# Autodesk Inventor assembly: Ensamble Herramienta
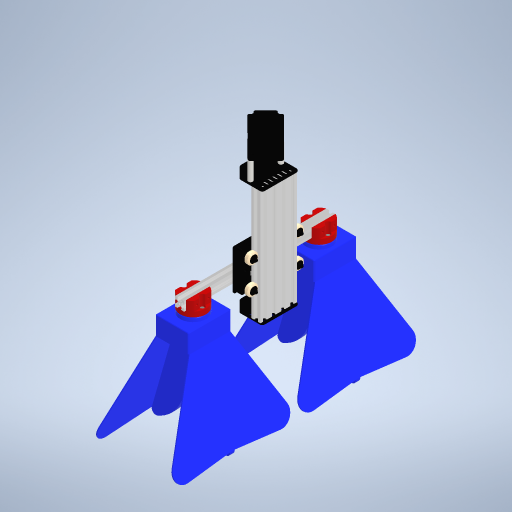
[picture p0: Inventor's stored thumbnail of the model, 512x512]
Saved by Autodesk Inventor 2024.2 (Build 282272000, 272)
## iProperties
Created: 2023-11-07
Part Number: Ensamble Herramienta
Document SubType Name: Assembly
Designer: juanp
Author: juanp
## Documents named in this file (9)
- C:\Users\jp.reyesf\OneDrive - Universidad de los andes\Uniandes\GPR Portable\Actuador\Ensamble Herramienta.iam
- C:\Users\jp.reyesf\OneDrive - Universidad de los andes\Uniandes\GPR Portable\Actuador\Antenas\Antena PowerLog.ipt
- C:\Users\jp.reyesf\OneDrive - Universidad de los andes\Uniandes\GPR Portable\Actuador\Acople Antena - Motor.ipt
- C:\Users\jp.reyesf\OneDrive - Universidad de los andes\Uniandes\GPR Portable\Actuador\VSLOT 2020 actuador.ipt
- C:\Users\jp.reyesf\OneDrive - Universidad de los andes\Uniandes\GPR Portable\Estructural\Tornillos y Tuercas\M5 x 10.ipt
- C:\Users\jp.reyesf\OneDrive - Universidad de los andes\Uniandes\GPR Portable\Estructural\Tornillos y Tuercas\T NUT M5 2020S\T NUT M5 2020S.ipt
- C:\Users\jp.reyesf\OneDrive - Universidad de los andes\Uniandes\GPR Portable\Actuador\Espaciador Actuador - Antenas.ipt
- C:\Users\jp.reyesf\OneDrive - Universidad de los andes\Uniandes\GPR Portable\Actuador\Actuador Lineal NEMA23\Actuador sin carro.iam
- C:\Users\jp.reyesf\OneDrive - Universidad de los andes\Uniandes\GPR Portable\Actuador\Actuador Lineal NEMA23\Carro.iam
## Components (24 placed, 8 different names)
1. Antena PowerLog:1 — Flush:4, Flush:5, Mate:27, Mate:28, Mate:30
2. Antena PowerLog:2 — Flush:4, Flush:5, Mate:27, Mate:29
3. Acople Antena - Motor:3 — Mate:28, Flush:6, Mate:30, Mate:34, Mate:35, Mate:36, Mate:37
4. Acople Antena - Motor:4 — Mate:29, Flush:6, Mate:31, Mate:32, Mate:33, Mate:38, Mate:39, Mate:40, Mate:41, Mate:42
5. VSLOT 2020 actuador:2 — Mate:31, Mate:32, Mate:33, Mate:44, Mate:50, Mate:51, Mate:52
6. M5 x 10:1 — Flush:8, Flush:9, Mate:36
7. M5 x 10:2 — Flush:9, Flush:13, Mate:34
8. M5 x 10:3 — Flush:7, Flush:8, Mate:37
9. M5 x 10:4 — Flush:7, Mate:35
10. M5 x 10:5 — Flush:10, Flush:11, Flush:12, Mate:40
11. M5 x 10:6 — Flush:11, Mate:39
12. M5 x 10:7 — Flush:10, Flush:13, Mate:38
13. M5 x 10:8 — Flush:12, Mate:41, Mate:42
14. T NUT M5 2020S:1 — Flush:14, Flush:15, Flush:16, Mate:45
15. T NUT M5 2020S:2 — Flush:14, Mate:46
16. Espaciador Actuador - Antenas:1 — Mate:44, Mate:45, Mate:46, Mate:47, Mate:48, Mate:50, Mate:52, Mate:53, Mate:54, Mate:55
17. T NUT M5 2020S:3 — Flush:16, Mate:47
18. T NUT M5 2020S:4 — Flush:15, Mate:48, Mate:51
19. Actuador sin carro:1 [sub-assembly] — Flush:20, Flush:21
20. Carro:1 [sub-assembly] — Mate:53, Mate:54, Mate:55, Mate:57, Mate:58, Mate:59, Mate:60, Mate:61, Flush:20, Flush:21
21. M5 x 10:9 — Flush:18, Flush:19, Mate:59
22. M5 x 10:10 — Flush:17, Mate:57
23. M5 x 10:11 — Flush:19, Mate:58, Mate:61
24. M5 x 10:12 — Flush:17, Flush:18, Mate:60
## Relationships (50: Mate 32, Flush 18)
- Flush:4: Antena PowerLog:1 ↔ Antena PowerLog:2
- Flush:5: Antena PowerLog:1 ↔ Antena PowerLog:2
- Mate:27 (275 mm): Antena PowerLog:1 ↔ Antena PowerLog:2
- Mate:28: Antena PowerLog:1 ↔ Acople Antena - Motor:3
- Mate:29: Antena PowerLog:2 ↔ Acople Antena - Motor:4
- Flush:6: Acople Antena - Motor:3 ↔ Acople Antena - Motor:4
- Mate:30: Antena PowerLog:1 ↔ Acople Antena - Motor:3
- Mate:31: Acople Antena - Motor:4 ↔ VSLOT 2020 actuador:2
- Mate:32: Acople Antena - Motor:4 ↔ VSLOT 2020 actuador:2
- Mate:33: Acople Antena - Motor:4 ↔ VSLOT 2020 actuador:2
- Flush:7: M5 x 10:3 ↔ M5 x 10:4
- Flush:8: M5 x 10:1 ↔ M5 x 10:3
- Flush:9: M5 x 10:1 ↔ M5 x 10:2
- Flush:10: M5 x 10:5 ↔ M5 x 10:7
- Flush:11: M5 x 10:5 ↔ M5 x 10:6
- Flush:12: M5 x 10:5 ↔ M5 x 10:8
- Flush:13: M5 x 10:2 ↔ M5 x 10:7
- Mate:34: Acople Antena - Motor:3 ↔ M5 x 10:2
- Mate:35: Acople Antena - Motor:3 ↔ M5 x 10:4
- Mate:36: Acople Antena - Motor:3 ↔ M5 x 10:1
- Mate:37: Acople Antena - Motor:3 ↔ M5 x 10:3
- Mate:38: Acople Antena - Motor:4 ↔ M5 x 10:7
- Mate:39: Acople Antena - Motor:4 ↔ M5 x 10:6
- Mate:40: Acople Antena - Motor:4 ↔ M5 x 10:5
- Mate:41: Acople Antena - Motor:4 ↔ M5 x 10:8
- Mate:42: Acople Antena - Motor:4 ↔ M5 x 10:8
- Flush:14: T NUT M5 2020S:1 ↔ T NUT M5 2020S:2
- Flush:15: T NUT M5 2020S:1 ↔ T NUT M5 2020S:4
- Flush:16: T NUT M5 2020S:1 ↔ T NUT M5 2020S:3
- Mate:44: VSLOT 2020 actuador:2 ↔ Espaciador Actuador - Antenas:1
- Mate:45: T NUT M5 2020S:1 ↔ Espaciador Actuador - Antenas:1
- Mate:46: T NUT M5 2020S:2 ↔ Espaciador Actuador - Antenas:1
- Mate:47: Espaciador Actuador - Antenas:1 ↔ T NUT M5 2020S:3
- Mate:48: Espaciador Actuador - Antenas:1 ↔ T NUT M5 2020S:4
- Mate:50: VSLOT 2020 actuador:2 ↔ Espaciador Actuador - Antenas:1
- Mate:51: VSLOT 2020 actuador:2 ↔ T NUT M5 2020S:4
- Mate:52: VSLOT 2020 actuador:2 ↔ Espaciador Actuador - Antenas:1
- Mate:53: Espaciador Actuador - Antenas:1 ↔ Carro:1
- Mate:54: Espaciador Actuador - Antenas:1 ↔ Carro:1
- Mate:55: Espaciador Actuador - Antenas:1 ↔ Carro:1
- Flush:17: M5 x 10:10 ↔ M5 x 10:12
- Flush:18: M5 x 10:9 ↔ M5 x 10:12
- Flush:19: M5 x 10:9 ↔ M5 x 10:11
- Mate:57: Carro:1 ↔ M5 x 10:10
- Mate:58: Carro:1 ↔ M5 x 10:11
- Mate:59: Carro:1 ↔ M5 x 10:9
- Mate:60: Carro:1 ↔ M5 x 10:12
- Mate:61: Carro:1 ↔ M5 x 10:11
- Flush:20: Actuador sin carro:1 ↔ Carro:1
- Flush:21: Actuador sin carro:1 ↔ Carro:1
